# Autodesk Inventor assembly: back
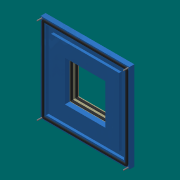
[picture p0: Inventor's stored thumbnail of the model, 180x180]
Saved by Autodesk Inventor 2016 (Build 200138000, 138)
## iProperties
Created: 2015-10-19
Part Number: back
Document SubType Name: Assembly
Designer: Sawaiz
Author: Sawaiz
## Documents named in this file (6)
- C:\Users\Sawaiz\OneDrive\projects\modularRICH\frame\back.iam
- C:\Users\Sawaiz\OneDrive\projects\modularRICH\frame\back.ipt
- C:\Users\Sawaiz\OneDrive\projects\modularRICH\frame\frontBackORing.ipt
- C:\Users\Sawaiz\OneDrive\projects\modularRICH\frame\sensorHolder.iam
- C:\Users\Sawaiz\OneDrive\projects\modularRICH\frame\0x0.5flatPhilips.ipt
- C:\Users\Sawaiz\OneDrive\projects\modularRICH\modularRICH.xlsx
## Components (8 placed, 4 different names)
1. back:1 — Mate:1, Mate:2, Mate:4, Flush:3, Flush:4, Mate:5, Mate:6, Flush:5, Mate:7, Mate:8, Mate:9, Flush:6, Flush:7, Flush:8
2. frontBackORing:1 — Mate:1, Mate:2, Mate:5
3. sensorHolder:1 [sub-assembly] — Mate:3, Flush:1, Flush:2, Flush:4
4. sensorHolder:2 [sub-assembly] — Mate:3, Flush:1, Flush:2, Mate:4, Flush:3
5. 0x0.5flatPhilips:1 — Mate:6, Flush:5
6. 0x0.5flatPhilips:2 — Mate:7, Flush:8
7. 0x0.5flatPhilips:3 — Mate:8, Flush:7
8. 0x0.5flatPhilips:4 — Mate:9, Flush:6
## Relationships (17: Mate 9, Flush 8)
- Mate:1: back:1 ↔ frontBackORing:1
- Mate:2: back:1 ↔ frontBackORing:1
- Mate:3: sensorHolder:1 ↔ sensorHolder:2
- Flush:1: sensorHolder:1 ↔ sensorHolder:2
- Flush:2: sensorHolder:1 ↔ sensorHolder:2
- Mate:4: back:1 ↔ sensorHolder:2
- Flush:3 (12.7 mm): back:1 ↔ sensorHolder:2
- Flush:4 (12.7 mm): back:1 ↔ sensorHolder:1
- Mate:5: back:1 ↔ frontBackORing:1
- Mate:6: back:1 ↔ 0x0.5flatPhilips:1
- Flush:5: back:1 ↔ 0x0.5flatPhilips:1
- Mate:7: back:1 ↔ 0x0.5flatPhilips:2
- Mate:8: back:1 ↔ 0x0.5flatPhilips:3
- Mate:9: back:1 ↔ 0x0.5flatPhilips:4
- Flush:6: back:1 ↔ 0x0.5flatPhilips:4
- Flush:7: back:1 ↔ 0x0.5flatPhilips:3
- Flush:8: back:1 ↔ 0x0.5flatPhilips:2
## Named parameters: acrylicThickness = 6.35 mm, aerogelThickness = 20 mm, height = 101.6 mm, width = 101.6 mm, depth = 101.6 mm, mirrorAngle = 5 deg, detectorWidth = 52 mm, detectorHeight = 52 mm, mirrorThickness = 3 mm, fresnelThickness = 0.1 mm, grooveDensity = 100, focalLength = 76.2 mm, ior = 1.49, centerThickness = 1.524 mm, fresnelAngle = 90 deg, fresnelEffectiveDiameter = 76.2 mm, mirrorSuppourtWidth = 38.1 mm, backGrooveBit = 4.8006 mm, sensorHolderWidth = 88.9 mm, sensorHolderHeight = 88.9 mm, sensorHolderSensorHeight = 53.975 mm, sensorHolderSensorWidth = 53.975 mm, oRingWidth = 3.175 mm, sensorHolderORingID = 203.2 mm, sensorHolderFlushORingID = 254 mm, frontBackORingID = 419.1 mm, topBottomHorizontalMirrorGroove = 12.7 mm, backMirrorGroove = 6.35 mm, mirrorGroove = 19.05 mm, compressionPercent = 40, fresnelChamfer = 6.35 mm, mirrorGrooveFillet = 6.35 mm, mirrorGrooveDrill = 6.35 mm, mirrorGrooveMill = 3.175 mm
